# Autodesk Inventor assembly: om_HIKOROBO_3.0
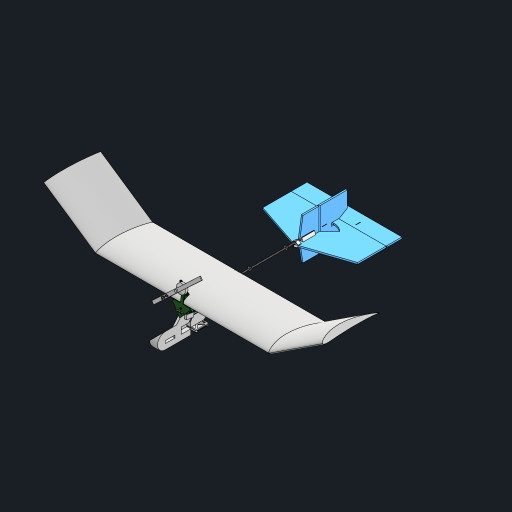
[picture p0: Inventor's stored thumbnail of the model, 512x512]
Saved by Autodesk Inventor 2023 (Build 270158000, 158)
## iProperties
Created: 2022-07-10
Part Number: om_HIKOROBO_3.0
Document SubType Name: Assembly
Designer: legot
Author: legot
## Documents named in this file (15)
- C:\Users\legot\Documents\Inventor\HIKOSAPO\1\om_HIKOROBO_3.0.iam
- C:\Users\legot\Documents\Inventor\HIKOSAPO\1\om_Body_3.0.ipt
- C:\Users\legot\Documents\Inventor\HIKOSAPO\1\MainRod.ipt
- C:\Users\legot\Documents\Inventor\HIKOSAPO\1\Drop\om_Drop_10g.iam
- C:\Users\legot\Documents\Inventor\HIKOSAPO\1\kiban.ipt
- C:\Users\legot\Documents\Inventor\HIKOSAPO\1\ServoMotor_8g.ipt
- C:\Users\legot\Documents\Inventor\HIKOSAPO\1\ServoMotor_Holder_V2.ipt
- C:\Users\legot\Documents\Inventor\HIKOSAPO\1\kibanHolder.ipt
- C:\Users\legot\Documents\Inventor\HIKOSAPO\1\WireHolder.ipt
- C:\Users\legot\Documents\Inventor\HIKOSAPO\1\Tail_Set.iam
- C:\Users\legot\Documents\Inventor\HIKOSAPO\1\MainWing_5.0.ipt
- C:\Users\legot\Documents\Inventor\HIKOSAPO\1\om_MotorMount_4.1.ipt
- C:\Users\legot\Documents\Inventor\HIKOSAPO\1\om_BackHolder_V4.ipt
- C:\Users\legot\Documents\Inventor\HIKOSAPO\1\MainMotor._Newipt.ipt
- C:\Users\legot\Documents\Inventor\HIKOSAPO\1\Propeller.ipt
## Components (16 placed, 14 different names)
1. om_Body_3.0:1 — メイト:5, メイト:6, メイト:8, メイト:9, メイト:11, フラッシュ:3, メイト:17, メイト:18, メイト:21, メイト:23, メイト:30, メイト:33, フラッシュ:8, フラッシュ:9, フラッシュ:10, フラッシュ:11, メイト:34, メイト:35, メイト:36, フラッシュ:12
2. MainRod:1 — メイト:5, メイト:26, メイト:27, メイト:28, フラッシュ:6, フラッシュ:7, メイト:31, メイト:32, フラッシュ:11, メイト:34
3. om_Drop_10g:1 [sub-assembly] — メイト:6, メイト:8, メイト:9
4. kiban:1 — メイト:19, 挿入:1, 挿入:2
5. ServoMotor_8g:1 — メイト:15, メイト:16, メイト:17
6. ServoMotor_8g:2 — メイト:13, メイト:14, メイト:18
7. ServoMotor_Holder_V2:1 — メイト:11, フラッシュ:3, メイト:13, メイト:14, メイト:15, メイト:16, フラッシュ:4
8. kibanHolder:1 — メイト:19, 挿入:1, メイト:21, 挿入:2, メイト:23
9. WireHolder:1 — メイト:26, メイト:27
10. Tail_Set:1 [sub-assembly] — メイト:28, フラッシュ:6, フラッシュ:7
11. MainWing_5.0:1 — メイト:30, フラッシュ:10, 正接:1
12. WireHolder:2 — メイト:31, メイト:32
13. om_MotorMount_4.1:1 — メイト:33, フラッシュ:8, フラッシュ:9, 正接:1, 挿入:3, 挿入:4
14. om_BackHolder_V4:1 — メイト:35, メイト:36, フラッシュ:12
15. MainMotor._Newipt:1 — 挿入:3, 挿入:4, 挿入:5
16. Propeller:1 — 挿入:5
## Relationships (39: Mate 24, Flush 9, Insert 5, Tangent 1)
- メイト:5 [Mate]: om_Body_3.0:1 ↔ MainRod:1
- メイト:6 [Mate]: om_Body_3.0:1 ↔ om_Drop_10g:1
- メイト:8 [Mate]: om_Body_3.0:1 ↔ om_Drop_10g:1
- メイト:9 [Mate]: om_Body_3.0:1 ↔ om_Drop_10g:1
- メイト:11 [Mate]: om_Body_3.0:1 ↔ ServoMotor_Holder_V2:1
- フラッシュ:3 [Flush]: om_Body_3.0:1 ↔ ServoMotor_Holder_V2:1
- メイト:13 [Mate]: ServoMotor_8g:2 ↔ ServoMotor_Holder_V2:1
- メイト:14 [Mate]: ServoMotor_8g:2 ↔ ServoMotor_Holder_V2:1
- メイト:15 [Mate]: ServoMotor_8g:1 ↔ ServoMotor_Holder_V2:1
- メイト:16 [Mate]: ServoMotor_8g:1 ↔ ServoMotor_Holder_V2:1
- メイト:17 [Mate]: om_Body_3.0:1 ↔ ServoMotor_8g:1
- メイト:18 [Mate]: om_Body_3.0:1 ↔ ServoMotor_8g:2
- メイト:19 [Mate]: kiban:1 ↔ kibanHolder:1
- 挿入:1 [Insert]: kiban:1 ↔ kibanHolder:1
- メイト:21 [Mate]: om_Body_3.0:1 ↔ kibanHolder:1
- 挿入:2 [Insert]: kiban:1 ↔ kibanHolder:1
- フラッシュ:4 [Flush]: ServoMotor_Holder_V2:1
- メイト:23 [Mate]: om_Body_3.0:1 ↔ kibanHolder:1
- メイト:26 [Mate]: MainRod:1 ↔ WireHolder:1
- メイト:27 [Mate]: MainRod:1 ↔ WireHolder:1
- メイト:28 [Mate]: MainRod:1 ↔ Tail_Set:1
- フラッシュ:6 [Flush]: MainRod:1 ↔ Tail_Set:1
- フラッシュ:7 [Flush]: MainRod:1 ↔ Tail_Set:1
- メイト:30 [Mate]: om_Body_3.0:1 ↔ MainWing_5.0:1
- メイト:31 [Mate]: MainRod:1 ↔ WireHolder:2
- メイト:32 [Mate]: MainRod:1 ↔ WireHolder:2
- メイト:33 [Mate]: om_Body_3.0:1 ↔ om_MotorMount_4.1:1
- フラッシュ:8 [Flush]: om_Body_3.0:1 ↔ om_MotorMount_4.1:1
- フラッシュ:9 [Flush]: om_Body_3.0:1 ↔ om_MotorMount_4.1:1
- フラッシュ:10 [Flush]: om_Body_3.0:1 ↔ MainWing_5.0:1
- 正接:1 [Tangent]: MainWing_5.0:1 ↔ om_MotorMount_4.1:1
- フラッシュ:11 [Flush]: om_Body_3.0:1 ↔ MainRod:1
- メイト:34 [Mate]: om_Body_3.0:1 ↔ MainRod:1
- メイト:35 [Mate]: om_Body_3.0:1 ↔ om_BackHolder_V4:1
- メイト:36 [Mate]: om_Body_3.0:1 ↔ om_BackHolder_V4:1
- フラッシュ:12 [Flush]: om_Body_3.0:1 ↔ om_BackHolder_V4:1
- 挿入:3 [Insert]: om_MotorMount_4.1:1 ↔ MainMotor._Newipt:1
- 挿入:4 [Insert]: om_MotorMount_4.1:1 ↔ MainMotor._Newipt:1
- 挿入:5 [Insert]: MainMotor._Newipt:1 ↔ Propeller:1
